# Autodesk Inventor assembly: Servo
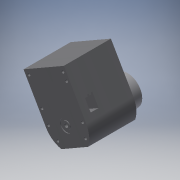
[picture p0: Inventor's stored thumbnail of the model, 180x180]
Saved by Autodesk Inventor 2016 (Build 200138000, 138)
## iProperties
Created: 2016-11-13
Part Number: Servo
Material: 一般
Document SubType Name: Assembly
Designer: Daisuke
Author: Daisuke
## Documents named in this file (4)
- C:\Users\Daisuke\Documents\GitHub\CAD\Hand\ver2\Servo.iam
- C:\Users\Daisuke\Documents\GitHub\CAD\Hand\ver2\FreeHorn.ipt
- C:\Users\Daisuke\Documents\GitHub\CAD\Hand\ver2\Gear20.ipt
- C:\Users\Daisuke\Documents\GitHub\CAD\Hand\ver2\Servo.ipt
## Components (3 placed, 3 different names)
1. FreeHorn:1 — 挿入:1, 挿入:2, 挿入:3, 挿入:4
2. Gear20:1 — 挿入:2, 挿入:3, 挿入:4
3. Servo:1 — 挿入:1
## Relationships (4: Insert 4)
- 挿入:1 [Insert]: FreeHorn:1 ↔ Servo:1
- 挿入:2 [Insert]: FreeHorn:1 ↔ Gear20:1
- 挿入:3 [Insert] (1 mm): FreeHorn:1 ↔ Gear20:1
- 挿入:4 [Insert] (1 mm): FreeHorn:1 ↔ Gear20:1
